# Autodesk Inventor assembly: ArduinoOnStilts
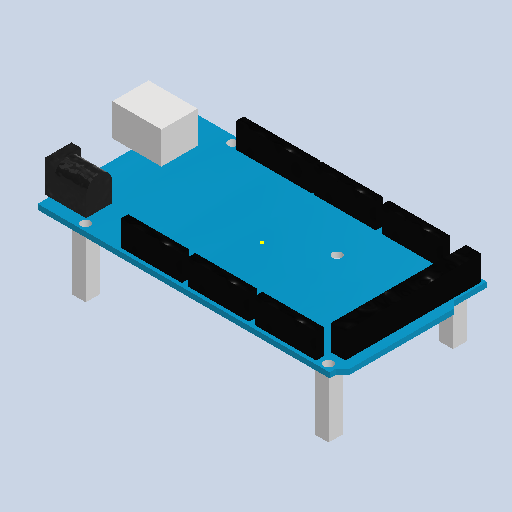
[picture p0: Inventor's stored thumbnail of the model, 512x512]
Saved by Autodesk Inventor 2023 (Build 270158000, 158)
## iProperties
Created: 2023-09-26
Part Number: ArduinoOnStilts
Document SubType Name: Assembly
Designer: Gage
Author: Gage
## Documents named in this file (3)
- C:\Users\Gage\OneDrive\Desktop\Autodesk Inventor\207\ArduinoOnStilts.iam
- C:\Users\Gage\OneDrive\Desktop\Autodesk Inventor\207\Arduino.ipt
- C:\Users\Gage\OneDrive\Desktop\Autodesk Inventor\207\ArduinoStilts.ipt
## Components (5 placed, 2 different names)
1. Arduino:1 — Mate:1, Mate:2, Mate:3, Mate:4
2. ArduinoStilts:1 — Mate:1
3. ArduinoStilts:2 — Mate:4
4. ArduinoStilts:3 — Mate:2
5. ArduinoStilts:4 — Mate:3
## Relationships (4: Mate 4)
- Mate:1: Arduino:1 ↔ ArduinoStilts:1
- Mate:2: Arduino:1 ↔ ArduinoStilts:3
- Mate:3: Arduino:1 ↔ ArduinoStilts:4
- Mate:4: Arduino:1 ↔ ArduinoStilts:2
